# Autodesk Inventor assembly: Satellite
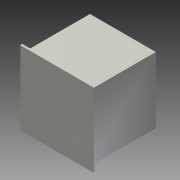
[picture p0: Inventor's stored thumbnail of the model, 180x180]
Saved by Autodesk Inventor 2015 SP1 (Build 190203100, 203)
## iProperties
Created: 2015-06-25
Part Number: Satellite
Document SubType Name: Assembly
Designer: Kartikye
Author: Kartikye
## Documents named in this file (4)
- C:\Users\Kartikye\Documents\GitHub\SASSat\Structure\Test1\Satellite.iam
- C:\Users\Kartikye\Documents\GitHub\SASSat\Structure\Test1\Base Plate.ipt
- C:\Users\Kartikye\Documents\GitHub\SASSat\Structure\Test1\Solar Panel PCB.ipt
- C:\Users\Kartikye\Documents\GitHub\SASSat\Structure\Test1\Top Blate.ipt
## Components (6 placed, 3 different names)
1. Base Plate:1 — Mate:1, Mate:2, Mate:3, Mate:4, Flush:3, Flush:4
2. Solar Panel PCB:1 — Mate:1, Mate:7, Mate:8, Flush:4, Mate:9, Flush:6
3. Solar Panel PCB:2 — Mate:2, Mate:5, Flush:1, Mate:7, Flush:3, Flush:5
4. Solar Panel PCB:3 — Mate:3, Mate:6, Flush:2, Mate:8
5. Solar Panel PCB:4 — Mate:4, Mate:5, Flush:1, Mate:6, Flush:2
6. Top Blate:1 — Mate:9, Flush:5, Flush:6
## Relationships (15: Mate 9, Flush 6)
- Mate:1: Base Plate:1 ↔ Solar Panel PCB:1
- Mate:2: Base Plate:1 ↔ Solar Panel PCB:2
- Mate:3: Base Plate:1 ↔ Solar Panel PCB:3
- Mate:4: Base Plate:1 ↔ Solar Panel PCB:4
- Mate:5: Solar Panel PCB:2 ↔ Solar Panel PCB:4
- Flush:1: Solar Panel PCB:2 ↔ Solar Panel PCB:4
- Mate:6: Solar Panel PCB:3 ↔ Solar Panel PCB:4
- Flush:2: Solar Panel PCB:3 ↔ Solar Panel PCB:4
- Mate:7: Solar Panel PCB:1 ↔ Solar Panel PCB:2
- Mate:8: Solar Panel PCB:1 ↔ Solar Panel PCB:3
- Flush:3 (3 mm): Base Plate:1 ↔ Solar Panel PCB:2
- Flush:4 (3 mm): Base Plate:1 ↔ Solar Panel PCB:1
- Mate:9: Solar Panel PCB:1 ↔ Top Blate:1
- Flush:5: Solar Panel PCB:2 ↔ Top Blate:1
- Flush:6: Solar Panel PCB:1 ↔ Top Blate:1
